# Autodesk Inventor assembly: Bat_contacts_v2_contact
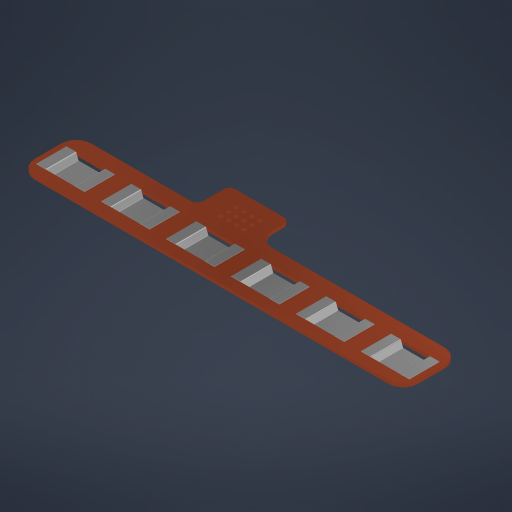
[picture p0: Inventor's stored thumbnail of the model, 512x512]
Saved by Autodesk Inventor 2024.3 (Build 283343010, 343A)
## iProperties
Created: 2025-05-13
Part Number: Bat_contacts_v2_contact
Document SubType Name: Assembly
Designer: David
Author: David
## Documents named in this file (3)
- C:\Users\David\Documents\FTAG\E-16\Batterie\Batterie_Konstruktion\E-16 Batterie\Bat_contacts_v2_contact.iam
- C:\Users\David\Documents\FTAG\E-16\Batterie\Batterie_Konstruktion\E-16 Batterie\bat_contacts_v2_plate_contact.ipt
- C:\Users\David\Documents\FTAG\E-16\Batterie\Batterie_Konstruktion\E-16 Batterie\bat_contacts_v2_contact.ipt
## Components (7 placed, 2 different names)
1. bat_contacts_v2_plate_contact:1 — Passend:1, Passend:2, Passend:3
2. bat_contacts_v2_contact:1 — Passend:1, Passend:2, Passend:3
3. bat_contacts_v2_contact:2
4. bat_contacts_v2_contact:3
5. bat_contacts_v2_contact:4
6. bat_contacts_v2_contact:5
7. bat_contacts_v2_contact:6
## Component patterns: (6 elements, first: bat_contacts_v2_contact:1)
## Relationships (3: Mate 3)
- Passend:1 [Mate]: bat_contacts_v2_plate_contact:1 ↔ bat_contacts_v2_contact:1
- Passend:2 [Mate]: bat_contacts_v2_plate_contact:1 ↔ bat_contacts_v2_contact:1
- Passend:3 [Mate]: bat_contacts_v2_plate_contact:1 ↔ bat_contacts_v2_contact:1
